# Autodesk Inventor assembly: Sensor_Halterung_Drehplatte
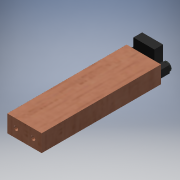
[picture p0: Inventor's stored thumbnail of the model, 180x180]
Saved by Autodesk Inventor 2018 (Build 220112000, 112)
## iProperties
Created: 2018-03-26
Part Number: Sensor_Halterung_Drehplatte
Material: Generisch
Document SubType Name: Assembly
Designer: Julian
Author: Julian
## Documents named in this file (4)
- C:\Users\Julian\Desktop\Schule\5AHME\Diplomarbeit\Git\fuettr_prototype\Mechanical\Inventorskizzen\Sensor_Halterung_Drehplatte.iam
- C:\Users\Julian\Documents\Inventor\Content Center Files\R2018\de-DE\DIN 96\DIN 96 - 2,5x8.ipt
- C:\Users\Julian\Desktop\Schule\5AHME\Diplomarbeit\Git\fuettr_prototype\Mechanical\Inventorskizzen\OPB732.ipt
- C:\Users\Julian\Desktop\Schule\5AHME\Diplomarbeit\Git\fuettr_prototype\Mechanical\Inventorskizzen\Sensor_Halterung_Drehplatte.ipt
## Components (4 placed, 3 different names)
1. DIN 96 2,5x8:1 — Starr:2
2. DIN 96 2,5x8:2 — Starr:3
3. OPB732:1 — Starr:1, Starr:2, Starr:3
4. Sensor_Halterung_Drehplatte:1 — Starr:1
## Relationships (3: WeldJoint 3)
- Starr:1 [WeldJoint]: OPB732:1 ↔ Sensor_Halterung_Drehplatte:1
- Starr:2 [WeldJoint]: DIN 96 2,5x8:1 ↔ OPB732:1
- Starr:3 [WeldJoint]: DIN 96 2,5x8:2 ↔ OPB732:1
